# Autodesk Inventor assembly: SteeringAssy
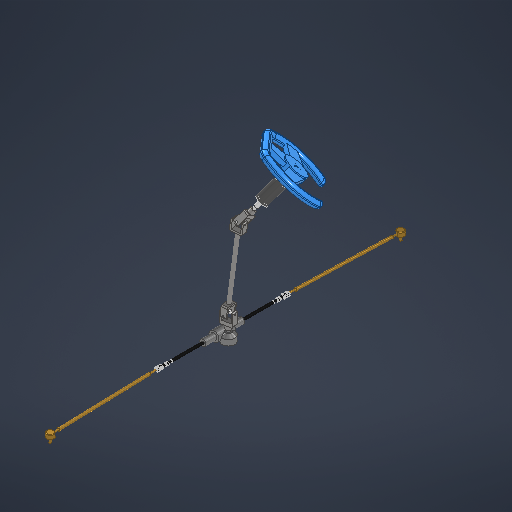
[picture p0: Inventor's stored thumbnail of the model, 512x512]
Saved by Autodesk Inventor 2026.2 (Build 302298010, 298A)
## iProperties
Created: 2026-07-06
Part Number: SteeringAssy
Document SubType Name: Assembly
Designer: tasle
Author: tasle
## Documents named in this file (11)
- C:\Users\tasle\Documents\PersonalProjects\FSAE\GOGO_FSAE_CAD\Steering\SteeringAssy.iam
- C:\Users\tasle\Documents\PersonalProjects\FSAE\GOGO_FSAE_CAD\Steering\Solid1.ipt
- C:\Users\tasle\Documents\PersonalProjects\FSAE\GOGO_FSAE_CAD\Steering\slider.ipt
- C:\Users\tasle\Documents\PersonalProjects\FSAE\GOGO_FSAE_CAD\Steering\tierod.ipt
- C:\Users\tasle\Documents\PersonalProjects\FSAE\GOGO_FSAE_CAD\Steering\Column.ipt
- C:\Users\tasle\Documents\PersonalProjects\FSAE\GOGO_FSAE_CAD\Steering\PinLarge.ipt
- C:\Users\tasle\Documents\PersonalProjects\FSAE\GOGO_FSAE_CAD\Steering\PinSmall.ipt
- C:\Users\tasle\Documents\PersonalProjects\FSAE\GOGO_FSAE_CAD\Steering\stick.ipt
- C:\Users\tasle\Documents\PersonalProjects\FSAE\GOGO_FSAE_CAD\Steering\adapter.ipt
- C:\Users\tasle\Documents\PersonalProjects\FSAE\GOGO_FSAE_CAD\Steering\hub.ipt
- C:\Users\tasle\Documents\PersonalProjects\FSAE\GOGO_FSAE_CAD\Steering\Solid1_1.ipt
## Components (14 placed, 10 different names)
1. Solid1:1 — Rotational:7, Rotational:10, Angle:1
2. slider:1 — Rotational:1, Rotational:2, Rotational:10, Angle:1
3. tierod:1 — Rotational:1
4. tierod:2 — Rotational:2
5. Column:1 — Rotational:3, Rotational:7
6. Column:2 — Rotational:4, Rotational:8
7. PinLarge:1 — Rotational:3, Rotational:6
8. PinSmall:1 — Rigid:1, Rotational:5
9. PinLarge:2 — Rotational:4, Rotational:5
10. PinSmall:2 — Rigid:2, Rotational:6
11. stick:1 — Rigid:1, Rigid:2
12. adapter:1 — Mate:1, Mate:2, Mate:3, Rotational:8, Rotational:9
13. hub:1 — Rotational:9
14. Solid1_1:1 — Mate:1, Mate:2, Mate:3
## Relationships (16: RevoluteJoint 10, Mate 3, WeldJoint 2, Angle 1)
- Rotational:1 [RevoluteJoint]: slider:1 ↔ tierod:1
- Rotational:2 [RevoluteJoint]: slider:1 ↔ tierod:2
- Rigid:1 [WeldJoint]: PinSmall:1 ↔ stick:1
- Rigid:2 [WeldJoint]: PinSmall:2 ↔ stick:1
- Rotational:3 [RevoluteJoint]: Column:1 ↔ PinLarge:1
- Rotational:4 [RevoluteJoint]: Column:2 ↔ PinLarge:2
- Rotational:5 [RevoluteJoint]: PinSmall:1 ↔ PinLarge:2
- Rotational:6 [RevoluteJoint]: PinLarge:1 ↔ PinSmall:2
- Rotational:7 [RevoluteJoint]: Solid1:1 ↔ Column:1
- Mate:1: adapter:1 ↔ Solid1_1:1
- Mate:2: adapter:1 ↔ Solid1_1:1
- Mate:3: adapter:1 ↔ Solid1_1:1
- Rotational:8 [RevoluteJoint]: Column:2 ↔ adapter:1
- Rotational:9 [RevoluteJoint] (35 mm): adapter:1 ↔ hub:1
- Rotational:10 [RevoluteJoint] (30 mm): Solid1:1 ↔ slider:1
- Angle:1 (0 deg): Solid1:1 ↔ slider:1
